# Autodesk Inventor assembly: FullFrame.004
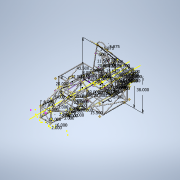
[picture p0: Inventor's stored thumbnail of the model, 180x180]
Saved by Autodesk Inventor 2021 (Build 250183000, 183)
## iProperties
Created: 2020-11-22
Part Number: FullFrame.004
Document SubType Name: Assembly
Designer: qv17m
_SolveAssemblyDoc: Frame Generator Solve Assembly
_Version: 25.0.0
Author: qv17m
## Documents named in this file (4)
- C:\Users\qv17m\Documents\Inventor\FSAE\FullCarV2.0\FullFrame.003\FullFrame.004.iam
- C:\Users\qv17m\Documents\Inventor\FSAE\FullCarV2.0\FullFrame.003\FrontFrame.003.ipt
- C:\Users\qv17m\Documents\Inventor\FSAE\FullCarV2.0\FullFrame.003\RearFrame.003.ipt
- C:\Users\qv17m\Documents\Inventor\FSAE\FullCarV2.0\FullFrame.003\FullFrame.004\Frame\Frame 1606066014995.iam
## Components (3 placed, 3 different names)
1. FrontFrame.003:1 — Mate:1
2. RearFrame.003:1 — Mate:1
3. Frame 1606066014995:1 [sub-assembly]
## Relationships (1: Mate 1)
- Mate:1: FrontFrame.003:1 ↔ RearFrame.003:1
